# Autodesk Inventor assembly: 射出_受け身
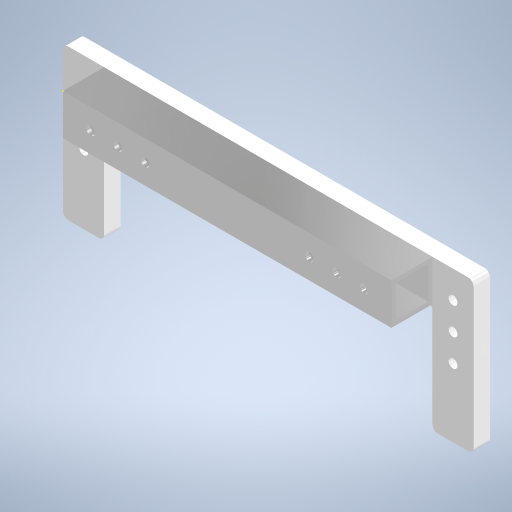
[picture p0: Inventor's stored thumbnail of the model, 512x512]
Saved by Autodesk Inventor 2023 (Build 270158000, 158)
## iProperties
Created: 2022-04-24
Part Number: 射出_受け身
Document SubType Name: Assembly
Designer: yuta
Author: yuta
## Documents named in this file (3)
- C:\Users\yuta\Documents\NHK\射出_受け身.iam
- C:\Users\yuta\Documents\NHK\射出_受け身.ipt
- C:\Users\yuta\Documents\NHK\射出_角柱12.ipt
## Components (2 placed, 2 different names)
1. 射出_受け身:1 — メイト:1, メイト:2, メイト:3, メイト:4, メイト:5
2. 射出_角柱12:1 — メイト:1, メイト:2, メイト:3, メイト:4, メイト:5
## Relationships (5: Mate 5)
- メイト:1 [Mate]: 射出_受け身:1 ↔ 射出_角柱12:1
- メイト:2 [Mate]: 射出_受け身:1 ↔ 射出_角柱12:1
- メイト:3 [Mate]: 射出_受け身:1 ↔ 射出_角柱12:1
- メイト:4 [Mate]: 射出_受け身:1 ↔ 射出_角柱12:1
- メイト:5 [Mate]: 射出_受け身:1 ↔ 射出_角柱12:1
